# Autodesk Inventor assembly: WeldedPlenumAssembly
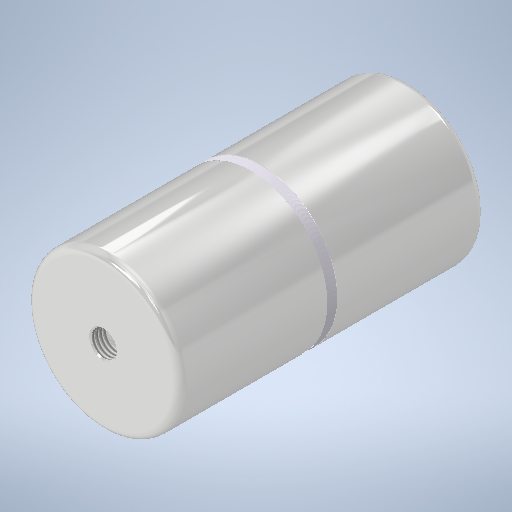
[picture p0: Inventor's stored thumbnail of the model, 512x512]
Saved by Autodesk Inventor 2025.2 (Build 292293000, 293)
## iProperties
Created: 2026-08-04
Part Number: WeldedPlenumAssembly
Document SubType Name: Weldment
Designer: Simon
Weld Material: Welded Aluminum-6061
Author: Simon
## Documents named in this file (3)
- C:\Users\Simon\Projects\MEng Electronics\Development of a Resistojet Thruster\3) Hardware\Resistojet Design\Prototype Design\Mechanical Drawings\WeldedPlenumAssembly.iam
- C:\Users\Simon\Projects\MEng Electronics\Development of a Resistojet Thruster\3) Hardware\Resistojet Design\Prototype Design\Mechanical Drawings\Plenum1.ipt
- C:\Users\Simon\Projects\MEng Electronics\Development of a Resistojet Thruster\3) Hardware\Resistojet Design\Prototype Design\Mechanical Drawings\Plenum2.ipt
## Components (2 placed, 2 different names)
1. Plenum1:1 — Mate:1, Mate:2
2. Plenum2:1 — Mate:1, Mate:2
## Relationships (2: Mate 2)
- Mate:1: Plenum1:1 ↔ Plenum2:1
- Mate:2: Plenum1:1 ↔ Plenum2:1
